# Autodesk Inventor assembly: Assembly1
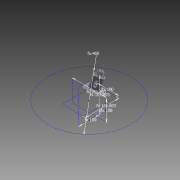
[picture p0: Inventor's stored thumbnail of the model, 180x180]
Saved by Autodesk Inventor 2014 (Build 180170000, 170)
## iProperties
Created: 2016-01-26
Part Number: Assembly1
Document SubType Name: Assembly
Designer: Justin B
Author: Justin B
## Documents named in this file (6)
- C:\Users\Justin B\Documents\aditest\ICO\Assembly1.iam
- C:\Users\Justin B\Documents\aditest\ICO\Frame.ipt
- C:\Users\Justin B\Documents\aditest\ICO\Shell.ipt
- C:\Users\Justin B\Documents\aditest\ICO\ShellFrame.ipt
- C:\Users\Justin B\Documents\aditest\ICO\RailGuide.ipt
- C:\Users\Justin B\Documents\aditest\ICO\Rail.ipt
## Components (7 placed, 5 different names)
1. Frame:1 — Mate:1, Mate:2, Flush:3
2. Shell:1 — Mate:1, Mate:2, Flush:1
3. ShellFrame:1 — Flush:1, Flush:4
4. RailGuide:1 — Flush:3
5. Rail:1 — Flush:4
6. Rail:2
7. Rail:3
## Component patterns: (3 elements, first: Rail:1)
## Relationships (5: Flush 3, Mate 2)
- Mate:1: Frame:1 ↔ Shell:1
- Mate:2: Frame:1 ↔ Shell:1
- Flush:1: Shell:1 ↔ ShellFrame:1
- Flush:3: Frame:1 ↔ RailGuide:1
- Flush:4: ShellFrame:1 ↔ Rail:1
